# Autodesk Inventor assembly: Para
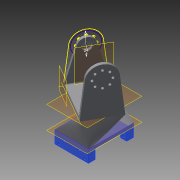
[picture p0: Inventor's stored thumbnail of the model, 180x180]
Saved by Autodesk Inventor 2015 (Build 190159000, 159)
## iProperties
Created: 2017-01-04
Part Number: Para
Document SubType Name: Assembly
Designer: Rudge-Top
Author: Rudge-Top
## Documents named in this file (4)
- C:\Users\Rudge-Top\Documents\RoboticArm\Inventor 2015\RotationLinks\Para.iam
- C:\Users\Rudge-Top\Documents\RoboticArm\Inventor 2015\Mounts\BaseMount.ipt
- C:\Users\Rudge-Top\Documents\RoboticArm\Inventor 2015\Mounts\Turnmount.ipt
- C:\Users\Rudge-Top\Documents\RoboticArm\Inventor 2015\RotationLinks\Parametric.ipt
## Components (3 placed, 3 different names)
1. BaseMount:1 — Mate:4, Mate:5, Mate:6
2. Turnmount:1 — Mate:1, Mate:2, Mate:3, Mate:7, Mate:8, Mate:9
3. Parametric:1 — Mate:1, Mate:2, Mate:3, Mate:4, Mate:5, Mate:6, Mate:7, Mate:8, Mate:9
## Relationships (9: Mate 9)
- Mate:1: Turnmount:1 ↔ Parametric:1
- Mate:2: Turnmount:1 ↔ Parametric:1
- Mate:3: Turnmount:1 ↔ Parametric:1
- Mate:4: BaseMount:1 ↔ Parametric:1
- Mate:5: BaseMount:1 ↔ Parametric:1
- Mate:6: BaseMount:1 ↔ Parametric:1
- Mate:7: Turnmount:1 ↔ Parametric:1
- Mate:8: Turnmount:1 ↔ Parametric:1
- Mate:9: Turnmount:1 ↔ Parametric:1
